# Autodesk Inventor assembly: Remote Assembly
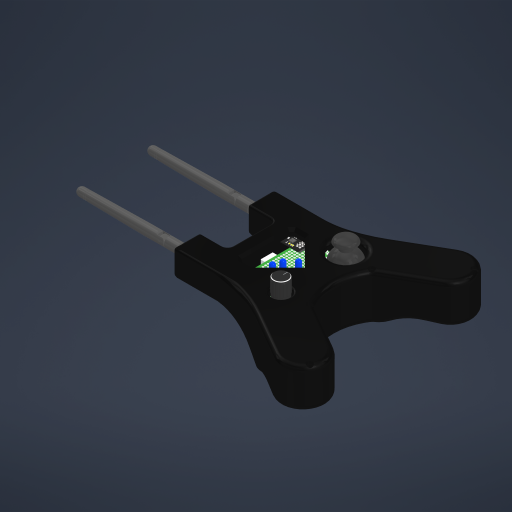
[picture p0: Inventor's stored thumbnail of the model, 512x512]
Saved by Autodesk Inventor 2024 (Build 280153000, 153)
## iProperties
Created: 2025-11-30
Part Number: Remote Assembly
Document SubType Name: Assembly
Designer: Vincent Larson
Author: Vincent Larson
## Documents named in this file (9)
- C:\Users\Vincent Larson\Downloads\Digital Ship Challenge\Digital Ship Challenge Remote\Remote Assembly.iam
- C:\Users\Vincent Larson\Downloads\Digital Ship Challenge\Digital Ship Challenge Remote\Arduino Uno\Arduino Uno.ipt
- C:\Users\Vincent Larson\Downloads\Digital Ship Challenge\Digital Ship Challenge Remote\NRF24L01L+Antenna\NRF24L01L+Antenna.iam
- C:\Users\Vincent Larson\Downloads\Digital Ship Challenge\Digital Ship Challenge Remote\Universal_board_70x90mm_31x26\Universal_board_70x90mm_31x26.iam
- C:\Users\Vincent Larson\Downloads\Digital Ship Challenge\Digital Ship Challenge Remote\KY-023_Joystick-Module\KY-023_Joystick-Module.iam
- C:\Users\Vincent Larson\Downloads\Digital Ship Challenge\Digital Ship Challenge Remote\SW2019 Rotary Encoder Knob Module\SW2019 Rotary Encoder Module.iam
- C:\Users\Vincent Larson\Downloads\Digital Ship Challenge\Digital Ship Challenge Remote\Blue LED\LED.ipt
- C:\Users\Vincent Larson\Downloads\Digital Ship Challenge\Digital Ship Challenge Remote\Remote Shell\Remote Shell Bottom.ipt
- C:\Users\Vincent Larson\Downloads\Digital Ship Challenge\Digital Ship Challenge Remote\Remote Shell\Remote Shell Top.ipt
## Components (13 placed, 8 different names)
1. Arduino Uno:1 — Mate:1
2. Universal_board_70x90mm_31x26:1 [sub-assembly] — Mate:1, Mate:2, Mate:3, Mate:4, Mate:5
3. NRF24L01L+Antenna:2 [sub-assembly] — Flush:1, Flush:2, Mate:2
4. NRF24L01L+Antenna:3 [sub-assembly] — Flush:1, Flush:2
5. KY-023_Joystick-Module:1 [sub-assembly] — Mate:3
6. SW2019 Rotary Encoder Module:1 [sub-assembly] — Mate:4
7. LED:1 — Flush:3, Mate:5
8. LED:2 — Flush:3, Flush:4
9. LED:3 — Flush:4, Flush:5
10. LED:4 — Flush:5, Flush:6
11. LED:5 — Flush:6
12. Remote Shell Bottom:1 — Mate:6, Flush:7, Flush:8
13. Remote Shell Top:1 — Mate:6, Flush:7, Flush:8
## Relationships (14: Flush 8, Mate 6)
- Mate:1: Arduino Uno:1 ↔ Universal_board_70x90mm_31x26:1
- Flush:1: NRF24L01L+Antenna:2 ↔ NRF24L01L+Antenna:3
- Flush:2: NRF24L01L+Antenna:2 ↔ NRF24L01L+Antenna:3
- Mate:2: Universal_board_70x90mm_31x26:1 ↔ NRF24L01L+Antenna:2
- Mate:3: Universal_board_70x90mm_31x26:1 ↔ KY-023_Joystick-Module:1
- Mate:4: Universal_board_70x90mm_31x26:1 ↔ SW2019 Rotary Encoder Module:1
- Flush:3: LED:1 ↔ LED:2
- Flush:4: LED:2 ↔ LED:3
- Flush:5: LED:3 ↔ LED:4
- Flush:6: LED:4 ↔ LED:5
- Mate:5: Universal_board_70x90mm_31x26:1 ↔ LED:1
- Mate:6: Remote Shell Bottom:1 ↔ Remote Shell Top:1
- Flush:7: Remote Shell Bottom:1 ↔ Remote Shell Top:1
- Flush:8: Remote Shell Bottom:1 ↔ Remote Shell Top:1
